# Autodesk Inventor assembly: Super Gantry
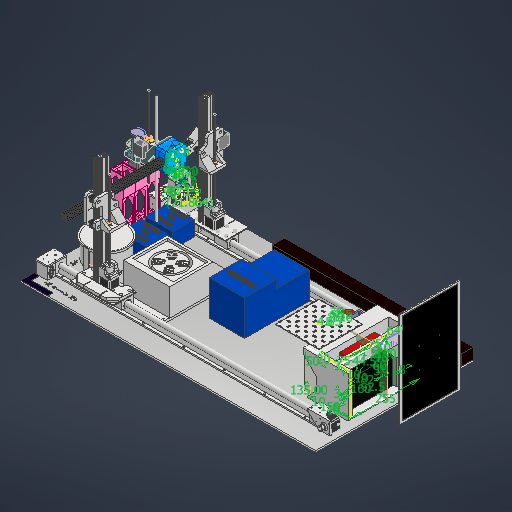
[picture p0: Inventor's stored thumbnail of the model, 512x512]
Saved by Autodesk Inventor 2025.1 (Build 291241000, 241)
## iProperties
Created: 2025-01-22
Part Number: Super Gantry
Document SubType Name: Assembly
Designer: jerem
Author: jerem
## Documents named in this file (20)
- C:\Users\jerem\Documents\GitHub\Perovskite-Automated-Synthesis-System\CAD\Gantry\Super Gantry.iam
- C:\Users\jerem\Documents\GitHub\Perovskite-Automated-Synthesis-System\CAD\Gantry\X Axis\X Axis.iam
- C:\Users\jerem\Documents\GitHub\Perovskite-Automated-Synthesis-System\CAD\Gantry\Z Axis\Z Axis.iam
- C:\Users\jerem\Documents\GitHub\Perovskite-Automated-Synthesis-System\CAD\Toolhead\Toolhead.iam
- C:\Users\jerem\Documents\GitHub\Perovskite-Automated-Synthesis-System\CAD\Camera\Camera Assembly.iam
- C:\Users\jerem\Documents\GitHub\Perovskite-Automated-Synthesis-System\CAD\Gripper\Redesign_GripperASSEM.iam
- C:\Users\jerem\Documents\GitHub\Perovskite-Automated-Synthesis-System\CAD\Gantry\Y Axis\Y Axis.iam
- C:\Users\jerem\Documents\GitHub\Perovskite-Automated-Synthesis-System\CAD\Pipette\PipetteStand.ipt
- C:\Users\jerem\Documents\GitHub\Perovskite-Automated-Synthesis-System\CAD\Non 3D Printed Parts\Objects\Cable Snake.ipt
- C:\Users\jerem\Documents\GitHub\Perovskite-Automated-Synthesis-System\CAD\Non 3D Printed Parts\Objects\HotPlate.ipt
- C:\Users\jerem\Documents\GitHub\Perovskite-Automated-Synthesis-System\CAD\Non 3D Printed Parts\Objects\TipDropoff.ipt
- C:\Users\jerem\Documents\GitHub\Perovskite-Automated-Synthesis-System\CAD\Non 3D Printed Parts\Objects\TipPickup.ipt
- C:\Users\jerem\Documents\GitHub\Perovskite-Automated-Synthesis-System\CAD\Gantry\Z Axis\Z Axis_MIR.iam
- C:\Users\jerem\Documents\GitHub\Perovskite-Automated-Synthesis-System\CAD\Non 3D Printed Parts\Monitor.ipt
- C:\Users\jerem\Documents\GitHub\Perovskite-Automated-Synthesis-System\CAD\vial carousel\Vial Carousel.iam
- C:\Users\jerem\Documents\GitHub\Perovskite-Automated-Synthesis-System\CAD\Spectrometer_Mount\Sample Infeed.iam
- C:\Users\jerem\Documents\GitHub\Perovskite-Automated-Synthesis-System\CAD\Spin-Chuck\Spincoater Assem.iam
- C:\Users\jerem\Documents\GitHub\Perovskite-Automated-Synthesis-System\CAD\vial carousel\Slide Tray.ipt
- C:\Users\jerem\Documents\GitHub\Perovskite-Automated-Synthesis-System\CAD\Ebox\Assembly1.iam
- C:\Users\jerem\Documents\GitHub\Perovskite-Automated-Synthesis-System\CAD\Pipette\SystemAssemV2.iam
## Components (21 placed, 19 different names)
1. X Axis:1 [sub-assembly] — Mate:25, Mate:26, Mate:27, Mate:34, Mate:41, Flush:7, Flush:8, Mate:42, Mate:44, Mate:45, Angle:2, Angle:3, Angle:4, Mate:48, Mate:54, Mate:59, Mate:60, Mate:61, Mate:62, Mate:63
2. Z Axis:1 [sub-assembly] — Mate:34, Mate:37, Angle:4, Flush:11
3. Toolhead:1 [sub-assembly] — Mate:8, Mate:9, Mate:10, Flush:1, Angle:1, Mate:36, Mate:57, Mate:58, Flush:10, Mate:64, Mate:65, Mate:66
4. Camera Assembly:1 [sub-assembly] — Mate:8, Mate:9, Mate:10
5. Redesign_GripperASSEM:1 [sub-assembly] — Mate:57, Mate:58, Flush:10
6. Y Axis:1 [sub-assembly] — Flush:1, Angle:1, Mate:36, Mate:37, Mate:49
7. PipetteStand:1 — Mate:26, Mate:28, Mate:29, Flush:2
8. PipetteStand:2 — Mate:25, Mate:28, Flush:2, Flush:3
9. PipetteStand:3 — Mate:27, Mate:29, Flush:3
10. Cable Snake:1 — Mate:41, Flush:7, Flush:8
11. HotPlate:1 — Mate:42, Mate:59
12. TipDropoff:1 — Mate:44, Angle:2
13. TipPickup:1 — Mate:45, Angle:3
14. Z Axis_MIR:1 [sub-assembly] — Mate:48, Mate:49, Flush:11
15. Monitor:1 — Mate:54
16. Vial Carousel:1 [sub-assembly] — Mate:60
17. Sample Infeed:1 [sub-assembly] — Mate:61
18. Spincoater Assem:1 [sub-assembly] — Mate:62
19. Slide Tray:1
20. Assembly1:1 [sub-assembly] — Mate:63
21. SystemAssemV2:1 [sub-assembly] — Mate:64, Mate:65, Mate:66
## Relationships (39: Mate 28, Flush 7, Angle 4)
- Mate:8: Toolhead:1 ↔ Camera Assembly:1
- Mate:9: Toolhead:1 ↔ Camera Assembly:1
- Mate:10: Toolhead:1 ↔ Camera Assembly:1
- Flush:1: Toolhead:1 ↔ Y Axis:1
- Mate:25: X Axis:1 ↔ PipetteStand:2
- Mate:26: X Axis:1 ↔ PipetteStand:1
- Mate:27: X Axis:1 ↔ PipetteStand:3
- Mate:28: PipetteStand:1 ↔ PipetteStand:2
- Mate:29: PipetteStand:1 ↔ PipetteStand:3
- Flush:2: PipetteStand:1 ↔ PipetteStand:2
- Flush:3: PipetteStand:2 ↔ PipetteStand:3
- Angle:1 (180 deg): Toolhead:1 ↔ Y Axis:1
- Mate:36: Toolhead:1 ↔ Y Axis:1
- Mate:34: X Axis:1 ↔ Z Axis:1
- Mate:37: Z Axis:1 ↔ Y Axis:1
- Mate:41: X Axis:1 ↔ Cable Snake:1
- Flush:7: X Axis:1 ↔ Cable Snake:1
- Flush:8: X Axis:1 ↔ Cable Snake:1
- Mate:42: X Axis:1 ↔ HotPlate:1
- Mate:44: X Axis:1 ↔ TipDropoff:1
- Mate:45: X Axis:1 ↔ TipPickup:1
- Angle:2 (180 deg): X Axis:1 ↔ TipDropoff:1
- Angle:3 (180 deg): X Axis:1 ↔ TipPickup:1
- Angle:4 (0 deg): X Axis:1 ↔ Z Axis:1
- Mate:48: X Axis:1 ↔ Z Axis_MIR:1
- Mate:49: Y Axis:1 ↔ Z Axis_MIR:1
- Mate:54: X Axis:1 ↔ Monitor:1
- Mate:57: Toolhead:1 ↔ Redesign_GripperASSEM:1
- Mate:58: Toolhead:1 ↔ Redesign_GripperASSEM:1
- Flush:10: Toolhead:1 ↔ Redesign_GripperASSEM:1
- Mate:59: X Axis:1 ↔ HotPlate:1
- Mate:60: X Axis:1 ↔ Vial Carousel:1
- Mate:61: X Axis:1 ↔ Sample Infeed:1
- Mate:62: X Axis:1 ↔ Spincoater Assem:1
- Mate:63: X Axis:1 ↔ Assembly1:1
- Flush:11: Z Axis:1 ↔ Z Axis_MIR:1
- Mate:64: Toolhead:1 ↔ SystemAssemV2:1
- Mate:65: Toolhead:1 ↔ SystemAssemV2:1
- Mate:66: Toolhead:1 ↔ SystemAssemV2:1
